# Autodesk Inventor assembly: buggy-assembly-group2
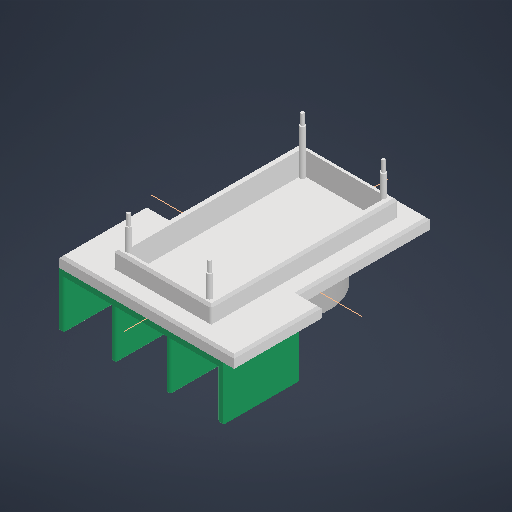
[picture p0: Inventor's stored thumbnail of the model, 512x512]
Saved by Autodesk Inventor 2026.1 (Build 301233000, 233)
## iProperties
Created: 2026-02-23
Part Number: buggy-assembly-group2
Document SubType Name: Assembly
Designer: ts2104
Author: ts2104
## Documents named in this file (4)
- C:\Users\dm2166\Downloads\buggy-assembly-group2.iam
- C:\Users\dm2166\Downloads\rubbish-container-group2.ipt
- H:\HWSYS\Desktop\Year 3\Inventor\crane-base-assembly.iam
- H:\HWSYS\Desktop\Year 3\Inventor\Buggy_Body_Wheel_Wells.ipt
## Components (3 placed, 3 different names)
1. rubbish-container-group2:1 — Mate:1, Mate:2, Mate:3, Flush:1
2. crane-base-assembly:1 [sub-assembly] — Mate:4
3. Buggy_Body_Wheel_Wells:1 — Mate:3, Flush:1, Mate:4
## Relationships (5: Mate 4, Flush 1)
- Mate:1: rubbish-container-group2:1
- Mate:2: rubbish-container-group2:1
- Mate:3: rubbish-container-group2:1 ↔ Buggy_Body_Wheel_Wells:1
- Flush:1: rubbish-container-group2:1 ↔ Buggy_Body_Wheel_Wells:1
- Mate:4: crane-base-assembly:1 ↔ Buggy_Body_Wheel_Wells:1
